# Autodesk Inventor assembly: Existing_Basement
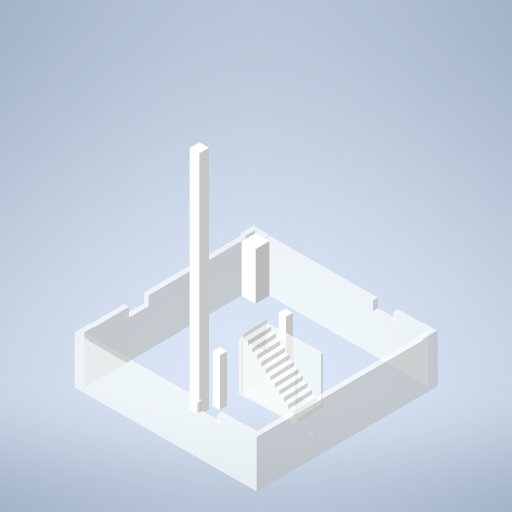
[picture p0: Inventor's stored thumbnail of the model, 512x512]
Saved by Autodesk Inventor 2024 (Build 280153000, 153)
## iProperties
Created: 2023-05-19
Part Number: Existing_Basement
Document SubType Name: Assembly
Designer: Tom
Author: Tom
## Documents named in this file (9)
- C:\Users\Tom\Documents\Tom_Levers_Public_Git_Repository\Inventor\Mobility\Basement\Existing_Basement.iam
- C:\Users\Tom\Documents\Tom_Levers_Public_Git_Repository\Inventor\Mobility\Basement\Exterior_Walls_Of_Existing_Basement.ipt
- C:\Users\Tom\Documents\Tom_Levers_Public_Git_Repository\Inventor\Mobility\Basement\Radon_And_Sump_Systems.ipt
- C:\Users\Tom\Documents\Tom_Levers_Public_Git_Repository\Inventor\Mobility\Basement\Chimney.ipt
- C:\Users\Tom\Documents\Tom_Levers_Public_Git_Repository\Inventor\Mobility\Basement\SW_Support_Column.ipt
- C:\Users\Tom\Documents\Tom_Levers_Public_Git_Repository\Inventor\Mobility\Basement\NE_Support_Column.ipt
- C:\Users\Tom\Documents\Tom_Levers_Public_Git_Repository\Inventor\Mobility\Basement\Stairs_Between_Existing_Basement_And_First_Floor.ipt
- C:\Users\Tom\Documents\Tom_Levers_Public_Git_Repository\Inventor\Mobility\Basement\Side_Wall_For_Existing_Stairwell.ipt
- C:\Users\Tom\Documents\Tom_Levers_Public_Git_Repository\Inventor\Mobility\Basement\Rear_Wall_For_Existing_Stairwell.ipt
## Components (9 placed, 8 different names)
1. Exterior_Walls_Of_Existing_Basement:1 — Mate:1, Flush:1, Flush:2, Mate:2, Flush:3, Flush:4, Mate:3, Flush:5, Flush:7, Mate:6, Mate:8, Mate:9, Flush:15, Flush:16, Flush:17, Mate:13
2. Radon_And_Sump_Systems:1 — Mate:1, Flush:1, Flush:2
3. Chimney:1 — Mate:2, Flush:3, Flush:4
4. SW_Support_Column:1 — Mate:3, Flush:5, Flush:15
5. NE_Support_Column:1 — Flush:7, Flush:17, Mate:13
6. Stairs_Between_Existing_Basement_And_First_Floor:1 — Mate:6, Mate:8, Mate:9, Mate:10, Flush:9, Flush:10, Mate:11, Flush:11, Flush:12, Mate:12, Flush:14, Flush:16
7. Side_Wall_For_Existing_Stairwell:1 — Mate:10, Flush:9, Flush:10, Flush:13
8. Side_Wall_For_Existing_Stairwell:2 — Mate:11, Flush:11, Flush:12
9. Rear_Wall_For_Existing_Stairwell:1 — Mate:12, Flush:13, Flush:14
## Relationships (25: Flush 15, Mate 10)
- Mate:1: Exterior_Walls_Of_Existing_Basement:1 ↔ Radon_And_Sump_Systems:1
- Flush:1: Exterior_Walls_Of_Existing_Basement:1 ↔ Radon_And_Sump_Systems:1
- Flush:2: Exterior_Walls_Of_Existing_Basement:1 ↔ Radon_And_Sump_Systems:1
- Mate:2 (1397 mm): Exterior_Walls_Of_Existing_Basement:1 ↔ Chimney:1
- Flush:3 (3009.9 mm): Exterior_Walls_Of_Existing_Basement:1 ↔ Chimney:1
- Flush:4: Exterior_Walls_Of_Existing_Basement:1 ↔ Chimney:1
- Mate:3 (2006.6 mm): Exterior_Walls_Of_Existing_Basement:1 ↔ SW_Support_Column:1
- Flush:5 (3365.5 mm): Exterior_Walls_Of_Existing_Basement:1 ↔ SW_Support_Column:1
- Flush:7: Exterior_Walls_Of_Existing_Basement:1 ↔ NE_Support_Column:1
- Mate:6 (3143.6564 mm): Exterior_Walls_Of_Existing_Basement:1 ↔ Stairs_Between_Existing_Basement_And_First_Floor:1
- Mate:8 (1409.7 mm): Exterior_Walls_Of_Existing_Basement:1 ↔ Stairs_Between_Existing_Basement_And_First_Floor:1
- Mate:9 (3073.7556 mm): Exterior_Walls_Of_Existing_Basement:1 ↔ Stairs_Between_Existing_Basement_And_First_Floor:1
- Mate:10: Stairs_Between_Existing_Basement_And_First_Floor:1 ↔ Side_Wall_For_Existing_Stairwell:1
- Flush:9: Stairs_Between_Existing_Basement_And_First_Floor:1 ↔ Side_Wall_For_Existing_Stairwell:1
- Flush:10: Stairs_Between_Existing_Basement_And_First_Floor:1 ↔ Side_Wall_For_Existing_Stairwell:1
- Mate:11: Stairs_Between_Existing_Basement_And_First_Floor:1 ↔ Side_Wall_For_Existing_Stairwell:2
- Flush:11: Stairs_Between_Existing_Basement_And_First_Floor:1 ↔ Side_Wall_For_Existing_Stairwell:2
- Flush:12: Stairs_Between_Existing_Basement_And_First_Floor:1 ↔ Side_Wall_For_Existing_Stairwell:2
- Mate:12: Stairs_Between_Existing_Basement_And_First_Floor:1 ↔ Rear_Wall_For_Existing_Stairwell:1
- Flush:13: Side_Wall_For_Existing_Stairwell:1 ↔ Rear_Wall_For_Existing_Stairwell:1
- Flush:14: Stairs_Between_Existing_Basement_And_First_Floor:1 ↔ Rear_Wall_For_Existing_Stairwell:1
- Flush:15: Exterior_Walls_Of_Existing_Basement:1 ↔ SW_Support_Column:1
- Flush:16: Exterior_Walls_Of_Existing_Basement:1 ↔ Stairs_Between_Existing_Basement_And_First_Floor:1
- Flush:17 (3365.5 mm): Exterior_Walls_Of_Existing_Basement:1 ↔ NE_Support_Column:1
- Mate:13 (2120.9 mm): Exterior_Walls_Of_Existing_Basement:1 ↔ NE_Support_Column:1
